# Autodesk Inventor assembly: two-section-bellows-on-bearings
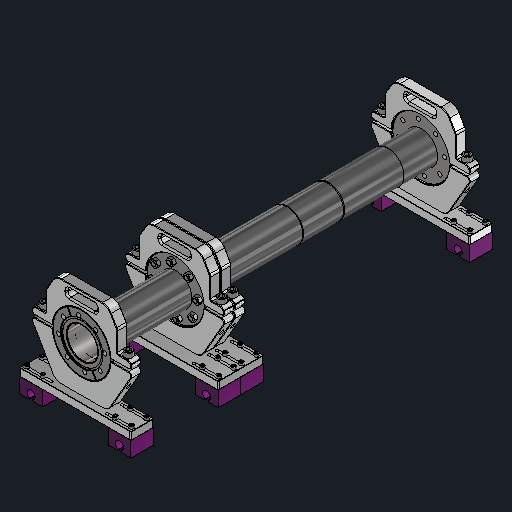
[picture p0: Inventor's stored thumbnail of the model, 512x512]
Saved by Autodesk Inventor 2027.1 (Build 311270010, 270A)
## iProperties
Part Number: two-section-bellows-on-bearings
Document SubType Name: Assembly
Designer: queezz
Author: queezz
## Documents named in this file (10)
- C:\Users\queezz\Dropbox\Drawings\pihti-cad\bellows-probe\two-section-bellows-on-bearings.iam
- C:\Users\queezz\Dropbox\Drawings\pihti-cad\bellows-probe\flange-camp-114.ipt
- C:\Users\queezz\Dropbox\Drawings\pihti-cad\bellows-probe\bellows_flange.ipt
- C:\Users\queezz\Dropbox\Drawings\pihti-cad\bellows-probe\instead-of-bellows.ipt
- C:\Users\queezz\Dropbox\Drawings\pihti-cad\bellows-probe\clamp-foot.ipt
- C:\Users\queezz\Dropbox\Drawings\pihti-cad\bellows-probe\clamp-foot-double.ipt
- C:\Users\queezz\Dropbox\Drawings\pihti-cad\bellows-probe\linearbearing-bolted.iam
- C:\Users\queezz\Dropbox\Drawings\pihti-cad\ContentCenter\Fastners\M8x45-HexCS.ipt
- C:\Users\queezz\Dropbox\Drawings\pihti-cad\ContentCenter\Fastners\m8-nut.ipt
- C:\Users\queezz\Dropbox\Drawings\pihti-cad\ContentCenter\Fastners\M10x30-SHCS.ipt
## Components (51 placed, 9 different names)
1. flange-camp-114:1
2. flange-camp-114:2 — Rotational:3
3. bellows_flange:1 — Middle flange bolt 1 - rigid, Middle flange bolt 2 - rigid, Middle flange bolt 3 - rigid, Middle flange bolt 4 - rigid, Middle flange bolt 5 - rigid, Middle flange bolt 6 - rigid, Middle flange bolt 7 - rigid, Middle flange bolt 8 - rigid
4. bellows_flange:2
5. instead-of-bellows:1
6. instead-of-bellows:2
7. clamp-foot:2
8. instead-of-bellows:3
9. instead-of-bellows:4
10. flange-camp-114:3 — Rigid:21
11. flange-camp-114:4
12. bellows_flange:3
13. bellows_flange:4 — Middle flange nut 1 - rigid, Middle flange nut 2 - rigid, Middle flange nut 3 - rigid, Middle flange nut 4 - rigid, Middle flange nut 5 - rigid, Middle flange nut 6 - rigid, Middle flange nut 7 - rigid, Middle flange nut 8 - rigid
14. instead-of-bellows:5
15. instead-of-bellows:6
16. clamp-foot:3
17. instead-of-bellows:7
18. instead-of-bellows:8
19. clamp-foot-double:1 — Rotational:3, Rigid:21, Central bearing 1 upright, Central bearing 3 upright
20. linearbearing-bolted:7 [sub-assembly]
21. linearbearing-bolted:1 [sub-assembly] — Central bearing 1 upright
22. linearbearing-bolted:2 [sub-assembly]
23. linearbearing-bolted:3 [sub-assembly] — Central bearing 3 upright
24. linearbearing-bolted:4 [sub-assembly]
25. linearbearing-bolted:5 [sub-assembly]
26. linearbearing-bolted:6 [sub-assembly]
27. linearbearing-bolted:8 [sub-assembly]
28. AS 1427 - Metric M8 x 45:1 — Middle flange bolt 2 - rigid
29. AS 1427 - Metric M8 x 45:2 — Middle flange bolt 3 - rigid
30. AS 1427 - Metric M8 x 45:3 — Middle flange bolt 4 - rigid
31. AS 1427 - Metric M8 x 45:4 — Middle flange bolt 5 - rigid
32. AS 1427 - Metric M8 x 45:5 — Middle flange bolt 6 - rigid
33. AS 1427 - Metric M8 x 45:6 — Middle flange bolt 7 - rigid
34. AS 1427 - Metric M8 x 45:7 — Middle flange bolt 8 - rigid
35. AS 1427 - Metric M8 x 45:8 — Middle flange bolt 1 - rigid
36. AS 1112 (2) - Metric M8  Type 5:1 — Middle flange nut 1 - rigid
37. AS 1112 (2) - Metric M8  Type 5:2 — Middle flange nut 2 - rigid
38. AS 1112 (2) - Metric M8  Type 5:3 — Middle flange nut 3 - rigid
39. AS 1112 (2) - Metric M8  Type 5:4 — Middle flange nut 4 - rigid
40. AS 1112 (2) - Metric M8  Type 5:5 — Middle flange nut 5 - rigid
41. AS 1112 (2) - Metric M8  Type 5:6 — Middle flange nut 6 - rigid
42. AS 1112 (2) - Metric M8  Type 5:7 — Middle flange nut 7 - rigid
43. AS 1112 (2) - Metric M8  Type 5:8 — Middle flange nut 8 - rigid
44. AS 1420 - Metric M10 x 30:17
45. AS 1420 - Metric M10 x 30:18
46. AS 1420 - Metric M10 x 30:19
47. AS 1420 - Metric M10 x 30:20
48. AS 1420 - Metric M10 x 30:21
49. AS 1420 - Metric M10 x 30:22
50. AS 1420 - Metric M10 x 30:23
51. AS 1420 - Metric M10 x 30:24
## Relationships (94: WeldJoint 33, Mate 31, Flush 25, Angle 4, RevoluteJoint 1)
- [Mate]: linearbearing-bolted:1 ↔ linearbearing-bolted:8
- [Flush]: flange-camp-114:1 ↔ clamp-foot:2
- [Mate]: flange-camp-114:1 ↔ clamp-foot:2
- [Mate]: flange-camp-114:1 ↔ clamp-foot:2
- [WeldJoint]: flange-camp-114:1 ↔ bellows_flange:2
- [WeldJoint]: flange-camp-114:1 ↔ AS 1420 - Metric M10 x 30:18
- [WeldJoint]: flange-camp-114:1 ↔ AS 1420 - Metric M10 x 30:17
- [Flush]: flange-camp-114:1 ↔ bellows_flange:2
- [Mate]: flange-camp-114:1 ↔ bellows_flange:2
- [Angle] (150 deg): flange-camp-114:1 ↔ bellows_flange:2
- [WeldJoint]: flange-camp-114:2 ↔ bellows_flange:1
- [WeldJoint]: flange-camp-114:2 ↔ AS 1420 - Metric M10 x 30:20
- [WeldJoint]: flange-camp-114:2 ↔ AS 1420 - Metric M10 x 30:19
- [Flush]: flange-camp-114:2 ↔ bellows_flange:1
- [Mate]: flange-camp-114:2 ↔ bellows_flange:1
- [Angle] (30 deg): flange-camp-114:2 ↔ bellows_flange:1
- [WeldJoint]: bellows_flange:1 ↔ instead-of-bellows:2
- [Mate] (-650 mm): bellows_flange:1 ↔ bellows_flange:2
- [WeldJoint]: bellows_flange:2 ↔ instead-of-bellows:1
- [Flush]: linearbearing-bolted:1 ↔ linearbearing-bolted:3
- [Mate]: linearbearing-bolted:1 ↔ linearbearing-bolted:4
- [Flush]: linearbearing-bolted:2 ↔ linearbearing-bolted:4
- [Flush]: linearbearing-bolted:2 ↔ linearbearing-bolted:4
- [Mate]: linearbearing-bolted:2 ↔ linearbearing-bolted:3
- [Flush]: clamp-foot:2 ↔ linearbearing-bolted:2
- [Flush]: clamp-foot:2 ↔ linearbearing-bolted:4
- [Flush]: clamp-foot:2 ↔ linearbearing-bolted:4
- [Flush]: clamp-foot:2 ↔ linearbearing-bolted:4
- [Mate]: instead-of-bellows:1 ↔ instead-of-bellows:2
- [Mate]: instead-of-bellows:1 ↔ instead-of-bellows:4
- [Mate] (-200 mm): instead-of-bellows:1 ↔ instead-of-bellows:4
- [Mate]: instead-of-bellows:2 ↔ instead-of-bellows:3
- [Mate]: instead-of-bellows:2 ↔ instead-of-bellows:3
- [Mate]: instead-of-bellows:3 ↔ instead-of-bellows:4
- [WeldJoint]: flange-camp-114:3 ↔ bellows_flange:4
- [WeldJoint]: flange-camp-114:3 ↔ AS 1420 - Metric M10 x 30:22
- [WeldJoint]: flange-camp-114:3 ↔ AS 1420 - Metric M10 x 30:21
- [Flush]: flange-camp-114:3 ↔ bellows_flange:4
- [Mate]: flange-camp-114:3 ↔ bellows_flange:4
- [Angle] (150 deg): flange-camp-114:3 ↔ bellows_flange:4
- [Mate]: flange-camp-114:4 ↔ clamp-foot:3
- [Mate]: flange-camp-114:4 ↔ clamp-foot:3
- [Flush]: flange-camp-114:4 ↔ clamp-foot:3
- [WeldJoint]: flange-camp-114:4 ↔ bellows_flange:3
- [WeldJoint]: flange-camp-114:4 ↔ AS 1420 - Metric M10 x 30:24
- [WeldJoint]: flange-camp-114:4 ↔ AS 1420 - Metric M10 x 30:23
- [Flush]: flange-camp-114:4 ↔ bellows_flange:3
- [Mate]: flange-camp-114:4 ↔ bellows_flange:3
- [Angle] (30 deg): flange-camp-114:4 ↔ bellows_flange:3
- [WeldJoint]: bellows_flange:3 ↔ instead-of-bellows:6
- [Mate] (-650 mm): bellows_flange:3 ↔ bellows_flange:4
- [WeldJoint]: bellows_flange:4 ↔ instead-of-bellows:5
- [Flush]: linearbearing-bolted:7 ↔ linearbearing-bolted:5
- [Flush]: clamp-foot:3 ↔ linearbearing-bolted:5
- [Mate]: linearbearing-bolted:5 ↔ linearbearing-bolted:8
- [Flush]: clamp-foot:3 ↔ linearbearing-bolted:5
- [Flush]: linearbearing-bolted:6 ↔ linearbearing-bolted:8
- [Flush]: linearbearing-bolted:6 ↔ linearbearing-bolted:8
- [Mate]: linearbearing-bolted:7 ↔ linearbearing-bolted:6
- [Mate]: clamp-foot:3 ↔ linearbearing-bolted:7
- [Flush]: clamp-foot:3 ↔ linearbearing-bolted:7
- [Flush]: clamp-foot:3 ↔ linearbearing-bolted:7
- [Mate]: instead-of-bellows:5 ↔ instead-of-bellows:6
- [Mate]: instead-of-bellows:5 ↔ instead-of-bellows:8
- [Mate] (-200 mm): instead-of-bellows:5 ↔ instead-of-bellows:8
- [Mate]: instead-of-bellows:6 ↔ instead-of-bellows:7
- [Mate]: instead-of-bellows:6 ↔ instead-of-bellows:7
- [Mate]: instead-of-bellows:7 ↔ instead-of-bellows:8
- [Mate]: linearbearing-bolted:3 ↔ linearbearing-bolted:6
- [Mate]: clamp-foot-double:1 ↔ linearbearing-bolted:8
- [Mate]: clamp-foot:2 ↔ linearbearing-bolted:4
- Rotational:3 [RevoluteJoint]: flange-camp-114:2 ↔ clamp-foot-double:1
- Rigid:21 [WeldJoint]: flange-camp-114:3 ↔ clamp-foot-double:1
- [Flush]: clamp-foot-double:1 ↔ linearbearing-bolted:1
- [Flush]: clamp-foot-double:1 ↔ linearbearing-bolted:3
- [Flush]: clamp-foot-double:1 ↔ linearbearing-bolted:6
- Middle flange bolt 1 - rigid [WeldJoint]: bellows_flange:1 ↔ AS 1427 - Metric M8 x 45:8
- Middle flange nut 1 - rigid [WeldJoint]: bellows_flange:4 ↔ AS 1112 (2) - Metric M8  Type 5:1
- Middle flange bolt 2 - rigid [WeldJoint]: bellows_flange:1 ↔ AS 1427 - Metric M8 x 45:1
- Middle flange nut 2 - rigid [WeldJoint]: bellows_flange:4 ↔ AS 1112 (2) - Metric M8  Type 5:2
- Middle flange bolt 3 - rigid [WeldJoint]: bellows_flange:1 ↔ AS 1427 - Metric M8 x 45:2
- Middle flange nut 3 - rigid [WeldJoint]: bellows_flange:4 ↔ AS 1112 (2) - Metric M8  Type 5:3
- Middle flange bolt 4 - rigid [WeldJoint]: bellows_flange:1 ↔ AS 1427 - Metric M8 x 45:3
- Middle flange nut 4 - rigid [WeldJoint]: bellows_flange:4 ↔ AS 1112 (2) - Metric M8  Type 5:4
- Middle flange bolt 5 - rigid [WeldJoint]: bellows_flange:1 ↔ AS 1427 - Metric M8 x 45:4
- Middle flange nut 5 - rigid [WeldJoint]: bellows_flange:4 ↔ AS 1112 (2) - Metric M8  Type 5:5
- Middle flange bolt 6 - rigid [WeldJoint]: bellows_flange:1 ↔ AS 1427 - Metric M8 x 45:5
- Middle flange nut 6 - rigid [WeldJoint]: bellows_flange:4 ↔ AS 1112 (2) - Metric M8  Type 5:6
- Middle flange bolt 7 - rigid [WeldJoint]: bellows_flange:1 ↔ AS 1427 - Metric M8 x 45:6
- Middle flange nut 7 - rigid [WeldJoint]: bellows_flange:4 ↔ AS 1112 (2) - Metric M8  Type 5:7
- Middle flange bolt 8 - rigid [WeldJoint]: bellows_flange:1 ↔ AS 1427 - Metric M8 x 45:7
- Middle flange nut 8 - rigid [WeldJoint]: bellows_flange:4 ↔ AS 1112 (2) - Metric M8  Type 5:8
- Central bearing 1 upright [Flush] (-35 mm): clamp-foot-double:1 ↔ linearbearing-bolted:1
- Central bearing 3 upright [Flush] (-35 mm): clamp-foot-double:1 ↔ linearbearing-bolted:3
## Named parameters: d53_d56 = 0 mm, d79_d113 = 0 mm, d80_d114 = 0 mm, d81_d55 = 0 mm, d82_d67 = 0 mm, d83_d68 = 150 deg, d84_d109 = 0 mm, d87_d111 = 0 mm, d88_d112 = 0 mm, d89_d69 = 0 mm, d90_d70 = 0 mm, d95_d75 = 30 deg, d96_d110 = 0 mm, d98_d71 = 0 mm, d99_d72 = 0 mm, d100_d73 = 0 mm, d101_d40 = -650 mm, d102_d41 = -135 mm, d103_d42 = -485 mm, d104_d22 = 0 mm, d105_d21 = 0 mm, d106_d36 = 0 mm, d107_d45 = 0 mm, d108_d74 = 0 mm, d115_d18 = 0 mm, d116_d37 = 0 mm, d118_d17 = 0 mm, d119_d19 = 0 mm, d126_d91 = 0 mm, d127_d24_d26 = 0 mm, d132_d61 = -200 mm, d133_d62 = 0 mm, d134_d63 = -200 mm, d135_d23 = 0 mm, d136_d57 = 0 mm, d137_d58 = 0 mm, d138_d59 = 0 mm, d139_d60 = -200 mm, d140_d64 = 0 mm, d141_d65 = 0 mm, d142_d66 = -200 mm
